# Autodesk Inventor assembly: kangarooSaberTooth
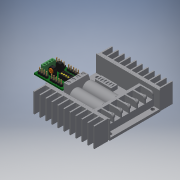
[picture p0: Inventor's stored thumbnail of the model, 180x180]
Saved by Autodesk Inventor 2017 (Build 210142000, 142)
## iProperties
Created: 2017-01-25
Part Number: kangarooSaberTooth
Document SubType Name: Assembly
Designer: Naga
Author: Naga
## Documents named in this file (3)
- C:\Users\Naga\Google Drive\IEEE CS\SoutheastCon2017\Cad\Electronics\kangarooSaberTooth.iam
- C:\Users\Naga\Google Drive\IEEE CS\SoutheastCon2017\Cad\Electronics\Sabertooth2x25A.ipt
- C:\Users\Naga\Google Drive\IEEE CS\SoutheastCon2017\Cad\Electronics\kangaroo x2_AP214.ipt
## Components (2 placed, 2 different names)
1. Sabertooth2x25A:1
2. kangaroo x2_AP214:1
## Relationships (3: Mate 2, Flush 1)
- [Mate]: Sabertooth2x25A:1 ↔ kangaroo x2_AP214:1
- [Mate] (3.175 mm): Sabertooth2x25A:1 ↔ kangaroo x2_AP214:1
- [Flush] (-0.635 mm): Sabertooth2x25A:1 ↔ kangaroo x2_AP214:1
## Named parameters: d10_d7 = 0 mm, d11_d8 = 3.175 mm, d12_d9 = -0.635 mm
